# Autodesk Inventor assembly: Playmobil Assembly
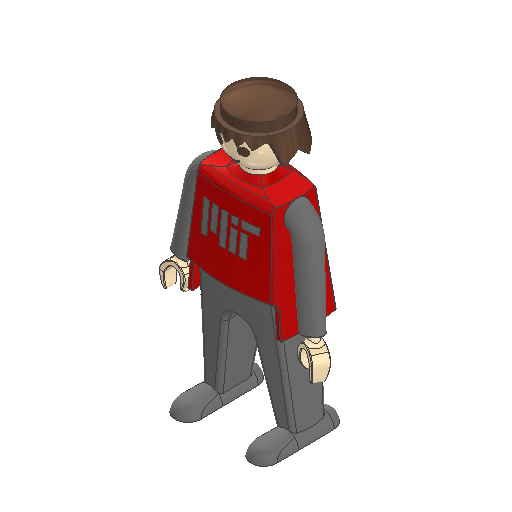
[picture p0: Inventor's stored thumbnail of the model, 512x512]
Saved by Autodesk Inventor 2026.2 (Build 302298000, 298)
## iProperties
Created: 2026-01-06
Part Number: Playmobil Assembly
Document SubType Name: Assembly
Designer: andyeske
Author: andyeske
## Documents named in this file (6)
- C:\Users\andyeske\Inventor\Playmobil Assembly.iam
- C:\Users\andyeske\Inventor\Playmobil 1.ipt
- C:\Users\andyeske\Inventor\Playmobil 2.ipt
- C:\Users\andyeske\Inventor\Playmobil 3.ipt
- C:\Users\andyeske\Inventor\Playmobil 4.ipt
- C:\Users\andyeske\Inventor\Playmobil 5.ipt
## Components (7 placed, 5 different names)
1. Playmobil 1:1 — Mate:1, Rotational:1, Rotational:2, Rotational:3, Rotational:6
2. Playmobil 2:1 — Mate:1, Rotational:1
3. Playmobil 3:1 — Rotational:2, Rotational:4
4. Playmobil 3:2 — Rotational:3, Rotational:5
5. Playmobil 4:1 — Rotational:4
6. Playmobil 4:2 — Rotational:5
7. Playmobil 5:1 — Rotational:6
## Relationships (7: RevoluteJoint 6, Mate 1)
- Mate:1: Playmobil 1:1 ↔ Playmobil 2:1
- Rotational:1 [RevoluteJoint]: Playmobil 1:1 ↔ Playmobil 2:1
- Rotational:2 [RevoluteJoint]: Playmobil 1:1 ↔ Playmobil 3:1
- Rotational:3 [RevoluteJoint]: Playmobil 1:1 ↔ Playmobil 3:2
- Rotational:4 [RevoluteJoint]: Playmobil 3:1 ↔ Playmobil 4:1
- Rotational:5 [RevoluteJoint]: Playmobil 3:2 ↔ Playmobil 4:2
- Rotational:6 [RevoluteJoint]: Playmobil 1:1 ↔ Playmobil 5:1
